# Autodesk Inventor assembly: gearbox
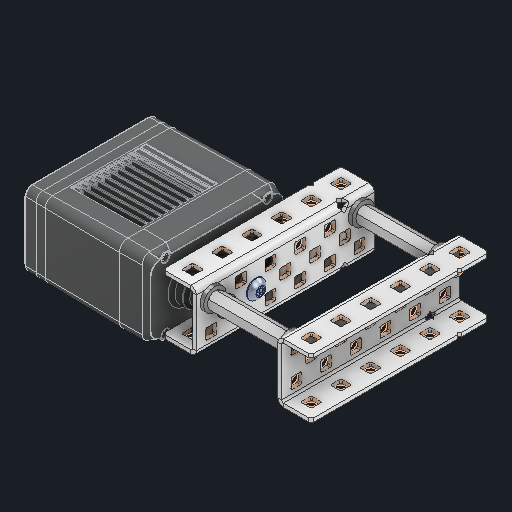
[picture p0: Inventor's stored thumbnail of the model, 512x512]
Saved by Autodesk Inventor 2025 (Build 290162000, 162)
## iProperties
Created: 2024-06-27
Part Number: gearbox
Document SubType Name: Assembly
Designer: Averey Ku
Author: Averey Ku
## Documents named in this file (8)
- D:\vex_robotics_high_stakes\hardware\cad\EARLY_SEASON\chassis\drivebay\gearbox.iam
- D:\vex_robotics_high_stakes\hardware\cad\VEX-CAD-Inventor\Electronics\Motors with Screws\SteelM-StarS.iam
- D:\vex_robotics_high_stakes\hardware\cad\VEX-CAD-Inventor\Electronics\Motors with Screws.iam
- D:\vex_robotics_high_stakes\hardware\cad\VEX-CAD-Inventor\Structure\C Channel\Aluminum 1x2x1\Alu C 1x2x1x6.ipt
- D:\vex_robotics_high_stakes\hardware\cad\VEX-CAD-Inventor\Structure\Standoff.ipt
- D:\vex_robotics_high_stakes\hardware\cad\VEX-CAD-Inventor\Motion\Spacers\Washer Steel\SWasher .375 OD x .062500.ipt
- D:\vex_robotics_high_stakes\hardware\cad\VEX-CAD-Inventor\Motion\Spacers\Washer Steel.ipt
- D:\vex_robotics_high_stakes\hardware\cad\VEX-CAD-Inventor\Structure\Standoff\Standoff 1.25.ipt
## Components (9 placed, 4 different names)
1. SteelM-StarS:1 [sub-assembly] — Insert:14, Mate:4
2. Alu C 1x2x1x6:1 — Insert:14, Mate:4
3. SWasher .375 OD x .062500:1 — Insert:10, Insert:13
4. SWasher .375 OD x .062500:2 — Insert:9
5. SWasher .375 OD x .062500:3 — Insert:12, Mate:3
6. SWasher .375 OD x .062500:4 — Insert:11
7. Standoff 1.25:1 — Insert:9, Insert:10
8. Standoff 1.25:2 — Insert:11, Insert:12
9. Alu C 1x2x1x6:2 — Insert:13, Mate:3
## Relationships (10: Insert 8, Mate 2)
- [Insert]: Alu C 1x2x1x6:1 ↔ SWasher .375 OD x .062500:2
- [Insert]: Alu C 1x2x1x6:1 ↔ SWasher .375 OD x .062500:4
- Insert:9: SWasher .375 OD x .062500:2 ↔ Standoff 1.25:1
- Insert:10: SWasher .375 OD x .062500:1 ↔ Standoff 1.25:1
- Insert:11: SWasher .375 OD x .062500:4 ↔ Standoff 1.25:2
- Insert:12: SWasher .375 OD x .062500:3 ↔ Standoff 1.25:2
- Insert:13: SWasher .375 OD x .062500:1 ↔ Alu C 1x2x1x6:2
- Mate:3: SWasher .375 OD x .062500:3 ↔ Alu C 1x2x1x6:2
- Insert:14: SteelM-StarS:1 ↔ Alu C 1x2x1x6:1
- Mate:4: SteelM-StarS:1 ↔ Alu C 1x2x1x6:1
